# Autodesk Inventor assembly: Assembly2
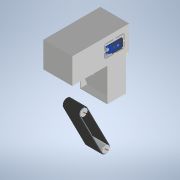
[picture p0: Inventor's stored thumbnail of the model, 180x180]
Saved by Autodesk Inventor 2022.2 (Build 262287000, 287)
## iProperties
Created: 2022-02-27
Part Number: Assembly2
Document SubType Name: Assembly
Designer: PRASHANTH
Author: PRASHANTH
## Documents named in this file (5)
- E:\BME\Autodesk Sample\Assembly2.iam
- E:\BME\Autodesk Sample\button unit.ipt
- E:\BME\Autodesk Sample\container unit.ipt
- E:\BME\Autodesk Sample\Arduino Mega main part.ipt
- E:\BME\Autodesk Sample\Assembly of Conveyor Belt.iam
## Components (4 placed, 4 different names)
1. button unit:1 — Mate:1, Flush:1, Mate:2, Mate:3, Flush:2
2. container unit:1 — Mate:3, Flush:2
3. Arduino Mega main part:1 — Mate:1, Flush:1, Mate:2
4. Assembly of Conveyor Belt:1 [sub-assembly]
## Relationships (5: Mate 3, Flush 2)
- Mate:1: button unit:1 ↔ Arduino Mega main part:1
- Flush:1 (8.5 mm): button unit:1 ↔ Arduino Mega main part:1
- Mate:2 (3 mm): button unit:1 ↔ Arduino Mega main part:1
- Mate:3: button unit:1 ↔ container unit:1
- Flush:2: button unit:1 ↔ container unit:1
